# Autodesk Inventor assembly: assem_linact_standalone_newfinger_v2_test
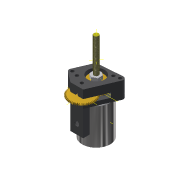
[picture p0: Inventor's stored thumbnail of the model, 180x180]
Saved by Autodesk Inventor 2014 (Build 180170000, 170)
## iProperties
Created: 2015-05-04
Part Number: assem_linact_standalone_newfinger_v2_test
Document SubType Name: Assembly
Designer: Martin
Author: Martin
## Documents named in this file (8)
- C:\Users\Martin\Dropbox\biohand-mec\biohand_v1\palm\assem_palm_linact.iam
- C:\Users\Martin\Dropbox\biohand-mec\biohand_v1\misc\m3_25_screw.ipt
- C:\Users\Martin\Dropbox\biohand-mec\biohand_v1\misc\m3_nut.ipt
- C:\Users\Martin\Dropbox\biohand-mec\biohand_v1\misc\servo_gear_2.ipt
- C:\Users\Martin\Dropbox\biohand-mec\biohand_v1\fingers\index\linact_top.ipt
- C:\Users\Martin\Dropbox\biohand-mec\biohand_v1\fingers\index\linact_base.ipt
- C:\Users\Martin\Dropbox\biohand-mec\biohand_v1\misc\motor_servo.ipt
- C:\Users\Martin\Dropbox\biohand-mec\biohand_v1\misc\servo_gear_1.ipt
## Components (7 placed, 7 different names)
1. m3_25_screw:1 — Insert:7
2. m3_nut:1 — Mate:5
3. servo_gear_2:1 — Mate:5, Insert:7
4. linact_top:1 — Mate:9, Mate:10, Mate:11, Insert:13
5. linact_base:1 — Mate:9, Mate:10, Mate:11, Insert:11
6. motor_servo:1 — Insert:11, Angle:3
7. servo_gear_1:1 — Insert:13
## Relationships (8: Mate 4, Insert 3, Angle 1)
- Mate:5: m3_nut:1 ↔ servo_gear_2:1
- Insert:7: m3_25_screw:1 ↔ servo_gear_2:1
- Mate:9: linact_top:1 ↔ linact_base:1
- Mate:10: linact_top:1 ↔ linact_base:1
- Mate:11: linact_top:1 ↔ linact_base:1
- Insert:11: linact_base:1 ↔ motor_servo:1
- Angle:3 (0 deg): motor_servo:1
- Insert:13 (0.3 mm): linact_top:1 ↔ servo_gear_1:1
